# Autodesk Inventor assembly: Assembly9
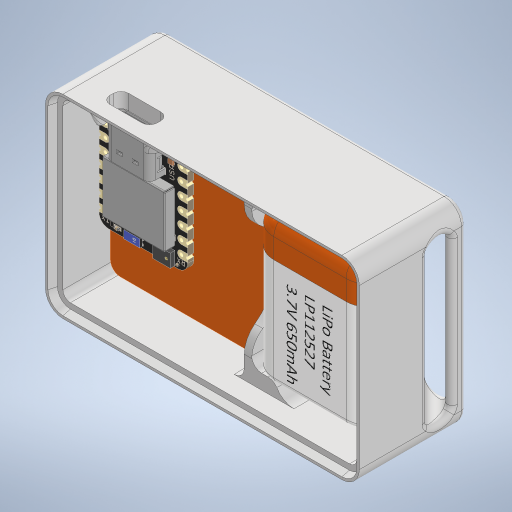
[picture p0: Inventor's stored thumbnail of the model, 512x512]
Saved by Autodesk Inventor 2024.3 (Build 283343000, 343)
## iProperties
Created: 2024-11-30
Part Number: Assembly9
Document SubType Name: Assembly
Designer: ASUS TUF
Author: ASUS TUF
## Documents named in this file (4)
- C:\Users\ASUS TUF\Documents\Inventor\ParkinsonDetection\Assembly9.iam
- C:\Users\ASUS TUF\Documents\Inventor\ParkinsonDetection\Case-V2.ipt
- C:\Users\ASUS TUF\Documents\Inventor\ParkinsonDetection\LP112527-3.7V650mAh\LP112527-3.7V650mAh\LP112527-3.7V650mAh.ipt
- C:\Users\ASUS TUF\Documents\Inventor\ParkinsonDetection\PCB.iam
## Components (3 placed, 3 different names)
1. Case-V2:1 — Mate:1, Mate:2, Mate:3, Mate:5, Tangent:1, Flush:1
2. LP112527-3.7V650mAh:1 — Mate:4, Mate:5, Tangent:1, Flush:1
3. PCB:1 [sub-assembly] — Mate:1, Mate:2, Mate:3, Mate:4
## Relationships (7: Mate 5, Tangent 1, Flush 1)
- Mate:1 (0.2 mm): Case-V2:1 ↔ PCB:1
- Mate:2: Case-V2:1 ↔ PCB:1
- Mate:3 (3 mm): Case-V2:1 ↔ PCB:1
- Mate:4 (2.1 mm): LP112527-3.7V650mAh:1 ↔ PCB:1
- Mate:5: Case-V2:1 ↔ LP112527-3.7V650mAh:1
- Tangent:1 (0.2 mm): Case-V2:1 ↔ LP112527-3.7V650mAh:1
- Flush:1 (0.2 mm): Case-V2:1 ↔ LP112527-3.7V650mAh:1
